# Autodesk Inventor assembly: underassy
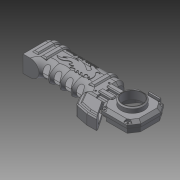
[picture p0: Inventor's stored thumbnail of the model, 180x180]
Saved by Autodesk Inventor 2018 (Build 220112000, 112)
## iProperties
Created: 2019-02-21
Part Number: underassy
Material: 一般
Document SubType Name: Assembly
Designer: ku_sk
Author: ku_sk
## Documents named in this file (4)
- E:\windows\Documents\Inventor\Content Center Files\bay shooter\parts\underassy.iam
- E:\windows\Documents\Inventor\Content Center Files\bay shooter\parts\undercover.ipt
- E:\windows\Documents\Inventor\Content Center Files\bay shooter\parts\dragon.ipt
- E:\windows\Documents\Inventor\Content Center Files\bay shooter\parts\dragon_MIR.ipt
## Components (3 placed, 3 different names)
1. undercover:1 — メイト:1, メイト:2, メイト:3, メイト:4
2. dragon:1 — 角度:1, メイト:4
3. dragon_MIR:1 — 角度:2
## Relationships (6: Mate 4, Angle 2)
- メイト:1 [Mate]: undercover:1
- メイト:2 [Mate]: undercover:1
- メイト:3 [Mate]: undercover:1
- 角度:1 [Angle] (0 deg): dragon:1
- メイト:4 [Mate] (-1 mm): undercover:1 ↔ dragon:1
- 角度:2 [Angle] (0 deg): dragon_MIR:1
